# Autodesk Inventor assembly: 2024_0121_MotorMount
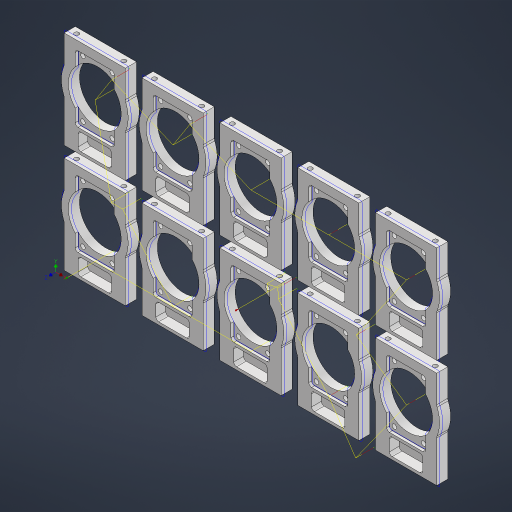
[picture p0: Inventor's stored thumbnail of the model, 512x512]
Saved by Autodesk Inventor 2024.2 (Build 282272000, 272)
## iProperties
Created: 2024-01-19
Part Number: 2024_0121_MotorMount
Document SubType Name: Assembly
Designer: Hanaoka
Author: Hanaoka
## Documents named in this file (2)
- G:\共有ドライブ\reRo\05_個人\hanaoka\inventor\CAMpath\2024_0121_MotorMount.iam
- G:\共有ドライブ\reRo\05_個人\hanaoka\inventor\DriveUnit\MotorMount_main.ipt
## Components (10 placed, 1 different names)
1. MotorMount_main:1 — メイト:1, メイト:2, 正接:1
2. MotorMount_main:2
3. MotorMount_main:3
4. MotorMount_main:4
5. MotorMount_main:5
6. MotorMount_main:6
7. MotorMount_main:7
8. MotorMount_main:8
9. MotorMount_main:9
10. MotorMount_main:10
## Component patterns: (10 elements, first: MotorMount_main:1)
## Relationships (3: Mate 2, Tangent 1)
- メイト:1 [Mate]: MotorMount_main:1
- メイト:2 [Mate]: MotorMount_main:1
- 正接:1 [Tangent]: MotorMount_main:1
